# Autodesk Inventor assembly: AC2DC_real
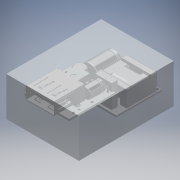
[picture p0: Inventor's stored thumbnail of the model, 180x180]
Saved by Autodesk Inventor 2018 (Build 220112000, 112)
## iProperties
Created: 2018-02-10
Part Number: AC2DC_real
Document SubType Name: Assembly
Designer: artur
Author: artur
## Documents named in this file (4)
- C:\Users\artur\Documents\projects\smartPowerStrip\CAD\Mechanical\AC2DC_real.iam
- C:\Users\artur\Documents\projects\smartPowerStrip\CAD\Mechanical\AC2DC_real.ipt
- C:\Users\artur\Documents\projects\smartPowerStrip\CAD\Mechanical\AC2DC_1.ipt
- C:\Users\artur\Documents\projects\smartPowerStrip\CAD\Mechanical\AC2DC_2.ipt
## Components (3 placed, 3 different names)
1. AC2DC_real:1 — Flush:1, Flush:2, Flush:3, Flush:4
2. AC2DC_1:1 — Flush:3, Flush:4
3. AC2DC_2:1 — Flush:1, Flush:2
## Relationships (4: Flush 4)
- Flush:1: AC2DC_real:1 ↔ AC2DC_2:1
- Flush:2: AC2DC_real:1 ↔ AC2DC_2:1
- Flush:3 (3.175 mm): AC2DC_real:1 ↔ AC2DC_1:1
- Flush:4: AC2DC_real:1 ↔ AC2DC_1:1
